# Autodesk Inventor assembly: Stewart-Base-KST-DS215
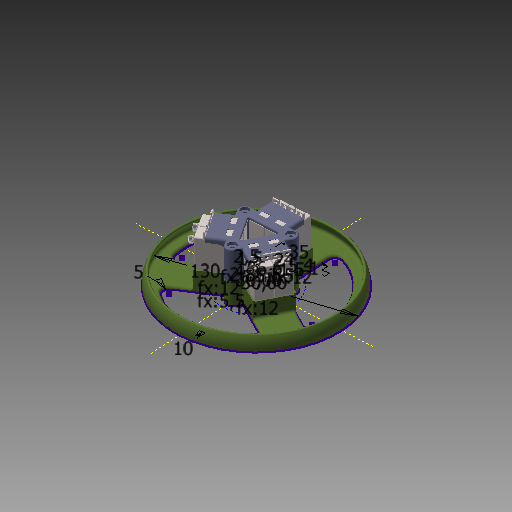
[picture p0: Inventor's stored thumbnail of the model, 512x512]
Saved by Autodesk Inventor 2018.2 (Build 222227000, 227)
## iProperties
Created: 2018-02-24
Part Number: Stewart-Base-KST-DS215
Material: Generisch
Document SubType Name: Assembly
Designer: JochenAlt
Author: JochenAlt
## Documents named in this file (3)
- D:\Projects\Donna\CAD\Stewart-Base.iam
- D:\Projects\Donna\CAD\Stewart-Platform-Base.ipt
- D:\Projects\Donna\CAD\Servo-KST-DS215MG.ipt
## Components (7 placed, 2 different names)
1. Stewart-Platform-Base-KST-DS215MG:1 — Passend:34, Passend:36, Passend:37, Passend:38, Passend:39, Passend:45, Passend:46, Passend:49, Passend:50, Passend:51, Passend:52, Passend:53, Passend:54, Passend:55, Passend:56, Passend:57, Passend:58, Passend:59, Passend:60
2. Servo-KST-DS215MG:1 — Passend:36, Passend:38, Passend:51
3. Servo-KST-DS215MG:2 — Passend:37, Passend:39, Passend:52
4. Servo-KST-DS215MG:3 — Passend:45, Passend:54, Passend:56
5. Servo-KST-DS215MG:4 — Passend:46, Passend:53, Passend:55
6. Servo-KST-DS215MG:5 — Passend:49, Passend:58, Passend:59
7. Servo-KST-DS215MG:6 — Passend:50, Passend:57, Passend:60
## Relationships (19: Mate 19)
- Passend:34 [Mate]: Stewart-Platform-Base-KST-DS215MG:1
- Passend:36 [Mate]: Stewart-Platform-Base-KST-DS215MG:1 ↔ Servo-KST-DS215MG:1
- Passend:37 [Mate]: Stewart-Platform-Base-KST-DS215MG:1 ↔ Servo-KST-DS215MG:2
- Passend:38 [Mate]: Stewart-Platform-Base-KST-DS215MG:1 ↔ Servo-KST-DS215MG:1
- Passend:39 [Mate]: Stewart-Platform-Base-KST-DS215MG:1 ↔ Servo-KST-DS215MG:2
- Passend:45 [Mate]: Stewart-Platform-Base-KST-DS215MG:1 ↔ Servo-KST-DS215MG:3
- Passend:46 [Mate]: Stewart-Platform-Base-KST-DS215MG:1 ↔ Servo-KST-DS215MG:4
- Passend:49 [Mate]: Stewart-Platform-Base-KST-DS215MG:1 ↔ Servo-KST-DS215MG:5
- Passend:50 [Mate]: Stewart-Platform-Base-KST-DS215MG:1 ↔ Servo-KST-DS215MG:6
- Passend:51 [Mate]: Stewart-Platform-Base-KST-DS215MG:1 ↔ Servo-KST-DS215MG:1
- Passend:52 [Mate]: Stewart-Platform-Base-KST-DS215MG:1 ↔ Servo-KST-DS215MG:2
- Passend:53 [Mate]: Stewart-Platform-Base-KST-DS215MG:1 ↔ Servo-KST-DS215MG:4
- Passend:54 [Mate]: Stewart-Platform-Base-KST-DS215MG:1 ↔ Servo-KST-DS215MG:3
- Passend:55 [Mate]: Stewart-Platform-Base-KST-DS215MG:1 ↔ Servo-KST-DS215MG:4
- Passend:56 [Mate]: Stewart-Platform-Base-KST-DS215MG:1 ↔ Servo-KST-DS215MG:3
- Passend:57 [Mate]: Stewart-Platform-Base-KST-DS215MG:1 ↔ Servo-KST-DS215MG:6
- Passend:58 [Mate]: Stewart-Platform-Base-KST-DS215MG:1 ↔ Servo-KST-DS215MG:5
- Passend:59 [Mate]: Stewart-Platform-Base-KST-DS215MG:1 ↔ Servo-KST-DS215MG:5
- Passend:60 [Mate]: Stewart-Platform-Base-KST-DS215MG:1 ↔ Servo-KST-DS215MG:6
